# Autodesk Inventor assembly: Sestava1
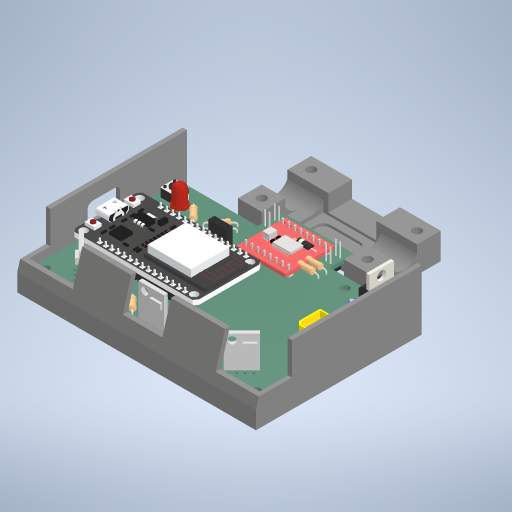
[picture p0: Inventor's stored thumbnail of the model, 512x512]
Saved by Autodesk Inventor 2024 (Build 280153000, 153)
## iProperties
Created: 2023-09-07
Part Number: Sestava1
Document SubType Name: Assembly
Designer: Simak
Author: Simak
## Documents named in this file (3)
- C:\Users\jaryj\Desktop\Škola\Mini sumo\RoboCop\- 3D -\wip\Sestava1.iam
- C:\Users\jaryj\Desktop\Škola\Mini sumo\RoboCop\- PCB -\SUMEC THT\sumec\sumec.ipt
- C:\Users\jaryj\Desktop\Škola\Mini sumo\RoboCop\- 3D -\wip\tělo.ipt
## Components (2 placed, 2 different names)
1. sumec:1 — Proti sobě:1, Vložit:1, Vložit:2
2. tělo:1 — Proti sobě:1, Vložit:1, Vložit:2
## Relationships (3: Insert 2, Mate 1)
- Proti sobě:1 [Mate]: sumec:1 ↔ tělo:1
- Vložit:1 [Insert]: sumec:1 ↔ tělo:1
- Vložit:2 [Insert]: sumec:1 ↔ tělo:1
